# Autodesk Inventor assembly: main_rename
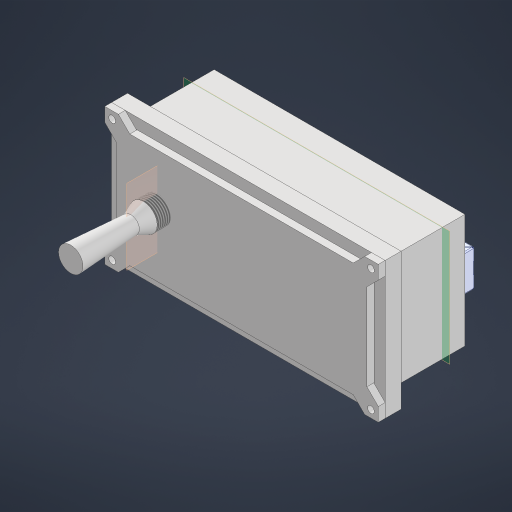
[picture p0: Inventor's stored thumbnail of the model, 512x512]
Saved by Autodesk Inventor 2024 (Build 280153000, 153)
## iProperties
Created: 2026-04-07
Part Number: main_rename
Document SubType Name: Assembly
Designer: schar
Author: schar
## Documents named in this file (5)
- C:\Users\schar\Desktop\MHIPS\models\tiles\2x1\lvl202x01_toggle\lvl202x01.iam
- C:\Users\schar\Desktop\MHIPS\models\racks\rack_C2x1.ipt
- C:\Users\schar\Desktop\MHIPS\models\tiles\2x1\lvl202x01_toggle\lvl202x01_toggle_body.ipt
- C:\Users\schar\Desktop\MHIPS\models\BusPlate\BusPlate.ipt
- C:\Users\schar\Desktop\MHIPS\models\switches\NKK_S1AL.ipt
## Components (4 placed, 4 different names)
1. rack_C2x1:1 — Flush:1
2. lvl202x01_toggle_body:1 — Flush:1, Mate:1, Mate:2, Mate:3
3. BusPlate:2 — Mate:1, Mate:2, Mate:3
4. NKK_S1AL:1
## Relationships (4: Mate 3, Flush 1)
- Flush:1: rack_C2x1:1 ↔ lvl202x01_toggle_body:1
- Mate:1 (0.2 mm): lvl202x01_toggle_body:1 ↔ BusPlate:2
- Mate:2 (3.16 mm): lvl202x01_toggle_body:1 ↔ BusPlate:2
- Mate:3: lvl202x01_toggle_body:1 ↔ BusPlate:2
